# Autodesk Inventor assembly: 조립품2
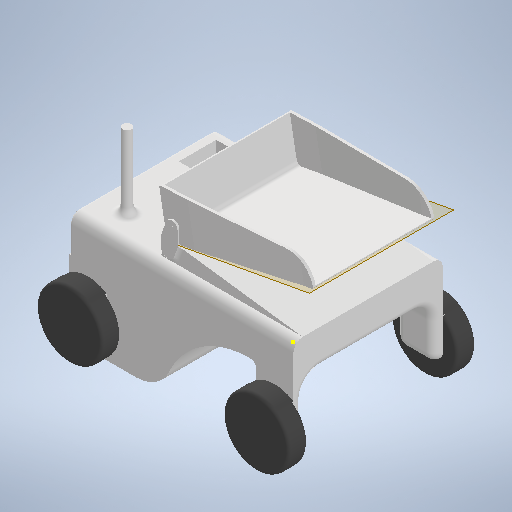
[picture p0: Inventor's stored thumbnail of the model, 512x512]
Saved by Autodesk Inventor 2025 (Build 290162010, 162A)
## iProperties
Created: 2024-06-17
Part Number: 조립품2
Document SubType Name: Assembly
Designer: user
Author: user
## Documents named in this file (3)
- J:\Inventor Files\RoProg24-1\조립품2.iam
- J:\Inventor Files\RoProg24-1\로봇팔본체.ipt
- J:\Inventor Files\RoProg24-1\basket.ipt
## Components (2 placed, 2 different names)
1. 로봇팔본체:1 — 플러쉬:2, 회전:1
2. basket:1 — 플러쉬:2, 회전:1
## Relationships (2: Flush 1, RevoluteJoint 1)
- 플러쉬:2 [Flush] (0.75 mm): 로봇팔본체:1 ↔ basket:1
- 회전:1 [RevoluteJoint]: 로봇팔본체:1 ↔ basket:1
